# Autodesk Inventor assembly: car
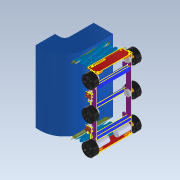
[picture p0: Inventor's stored thumbnail of the model, 180x180]
Saved by Autodesk Inventor 2022 (Build 260153000, 153)
## iProperties
Created: 2023-04-20
Part Number: car
Document SubType Name: Assembly
Designer: Johnny Jou
Author: Johnny Jou
## Documents named in this file (24)
- C:\Users\Johnny Jou\Documents\GitHub\Areo_Rider_Cabin\car\car.iam
- C:\Users\Johnny Jou\Documents\GitHub\Areo_Rider_Cabin\car\chassis_1_1\chassis_1_1-02.ipt
- C:\Users\Johnny Jou\Documents\GitHub\Areo_Rider_Cabin\car\chassis_1_1.ipt
- C:\Users\Johnny Jou\Documents\GitHub\Areo_Rider_Cabin\car\chassis_1_1\chassis_1_1-03.ipt
- C:\Users\Johnny Jou\Documents\GitHub\Areo_Rider_Cabin\car\chassis_1_2.ipt
- C:\Users\Johnny Jou\Documents\GitHub\Areo_Rider_Cabin\Expansion\link_2022.ipt
- C:\Users\Johnny Jou\Documents\GitHub\Areo_Rider_Cabin\Expansion\gasket.ipt
- C:\Users\Johnny Jou\Documents\GitHub\Areo_Rider_Cabin\car\car\機械便覽魔法師\軸承1.iam
- C:\Users\Johnny Jou\Documents\GitHub\Areo_Rider_Cabin\car\wheel_base_cover.ipt
- C:\Users\Johnny Jou\Documents\GitHub\Areo_Rider_Cabin\car\axle 4_20.ipt
- C:\Users\Johnny Jou\Documents\GitHub\Areo_Rider_Cabin\car\Coupling.ipt
- C:\Users\Johnny Jou\Documents\GitHub\Areo_Rider_Cabin\car\wheel.ipt
- C:\Users\Johnny Jou\Documents\GitHub\Areo_Rider_Cabin\car\外抓檔\25GA370.ipt
- C:\Users\Johnny Jou\Documents\GitHub\Areo_Rider_Cabin\Expansion\rod_2.ipt
- C:\Users\Johnny Jou\Documents\GitHub\Areo_Rider_Cabin\car\chassis_1_4.ipt
- C:\Users\Johnny Jou\Documents\GitHub\Areo_Rider_Cabin\car\motorbase_1.ipt
- C:\Users\Johnny Jou\Documents\GitHub\Areo_Rider_Cabin\car\motorbase_2.ipt
- C:\Users\Johnny Jou\Documents\GitHub\Areo_Rider_Cabin\car\motorbase_3.ipt
- C:\Users\Johnny Jou\Documents\GitHub\Areo_Rider_Cabin\car\motorbase_4.ipt
- C:\Users\Johnny Jou\Documents\GitHub\Areo_Rider_Cabin\car\外抓檔\GA12-N20 Motor-Complet.iam
- C:\Users\Johnny Jou\Documents\GitHub\Areo_Rider_Cabin\car\motorbase_5.ipt
- C:\Users\Johnny Jou\Documents\GitHub\Areo_Rider_Cabin\car\chassis_1_2_up.ipt
- C:\Users\Johnny Jou\Documents\GitHub\Areo_Rider_Cabin\car\chassis_1_3.ipt
- C:\Users\Johnny Jou\Documents\GitHub\Areo_Rider_Cabin\Airfoil & Nuzzle\nuzzle\nuzzle_v2_0327.ipt
## Components (76 placed, 22 different names)
1. chassis_1_1-02:1 — 齊平:1, 貼合:4, 貼合:5, 齊平:3, 貼合:6, 貼合:7, 貼合:46, 貼合:47, 貼合:48, 貼合:59, 貼合:60, 貼合:61, 貼合:68, 貼合:69, 貼合:70, 齊平:12, 齊平:21, 貼合:112, 貼合:113, 貼合:114, 貼合:115, 貼合:116, 齊平:32, 貼合:117, 齊平:33, 貼合:118, 貼合:119, 齊平:34, 貼合:120, 貼合:121, 齊平:35, 貼合:122
2. chassis_1_1-03:2 — 貼合:2, 貼合:3, 齊平:2, 貼合:43, 貼合:44, 貼合:45, 貼合:56, 貼合:57, 貼合:58, 貼合:71, 貼合:72, 貼合:73, 齊平:14, 齊平:18, 貼合:83, 貼合:84, 貼合:85, 貼合:86, 貼合:87, 貼合:88, 貼合:89, 貼合:90, 貼合:94, 貼合:96, 貼合:97, 貼合:103, 貼合:104, 貼合:105, 貼合:106, 貼合:107, 貼合:108, 貼合:109
3. chassis_1_2:1 — 齊平:1, 貼合:2, 貼合:3, 齊平:2, 貼合:4, 貼合:5, 插入:16, 貼合:8, 角度:7, 貼合:82, 齊平:11, 齊平:15
4. chassis_1_2:2 — 齊平:3, 貼合:6, 貼合:7, 插入:17, 貼合:9, 齊平:17, 齊平:20
5. link_2022:1 — 插入:1, 插入:3, 角度:1, 插入:17
6. link_2022:2 — 插入:1, 插入:2, 插入:7, 角度:2
7. link_2022:3 — 插入:2, 插入:4, 插入:6, 角度:2
8. link_2022:4 — 插入:3, 插入:4, 角度:1, 貼合:9, 貼合:80, 貼合:81
9. link_2022:5 — 插入:6, 角度:3, 插入:21
10. link_2022:6 — 插入:7, 角度:3, 貼合:110
11. link_2022:7 — 貼合:8, 插入:18
12. link_2022:8
13. link_2022:9
14. link_2022:10 — 插入:15
15. link_2022:11 — 貼合:111
16. link_2022:12 — 插入:22
17. gasket:1 — 插入:15, 插入:16
18. 軸承:2 [sub-assembly]
19. wheel_base_cover:2 — 貼合:43, 貼合:44, 貼合:45
20. axle 4_20:2
21. Coupling:2
22. wheel:2
23. 軸承:3 [sub-assembly]
24. wheel_base_cover:3 — 貼合:46, 貼合:47, 貼合:48
25. axle 4_20:3
26. Coupling:3
27. wheel:3
28. 軸承:4 [sub-assembly]
29. wheel_base_cover:4 — 貼合:59, 貼合:60, 貼合:61
30. axle 4_20:4
31. Coupling:4
32. wheel:4 — 齊平:36
33. Coupling:5 — 貼合:62, 貼合:63
34. wheel:5
35. 軸承:5 [sub-assembly]
36. wheel_base_cover:5 — 貼合:56, 貼合:57, 貼合:58
37. axle 4_20:5
38. Coupling:6
39. wheel:6
40. 25GA370:1 — 貼合:62, 貼合:63, 貼合:71, 貼合:72, 貼合:73
41. Coupling:7
42. wheel:7
43. 25GA370:2 — 貼合:68, 貼合:69, 貼合:70
44. rod_2:1 — 貼合:75, 貼合:76, 貼合:78, 貼合:79, 角度:7, 貼合:80, 貼合:81
45. 軸承:6 [sub-assembly] — 貼合:76
46. axle 4_20:8 — 貼合:75
47. 軸承:7 [sub-assembly] — 貼合:79
48. axle 4_20:9 — 貼合:78
49. gasket:2 — 插入:18
50. chassis_1_4:1 — 貼合:82, 齊平:11, 齊平:12, 齊平:13, 齊平:16, 齊平:19
51. chassis_1_4:2 — 齊平:19, 齊平:20, 齊平:21
52. chassis_1_4:3 — 齊平:16, 齊平:17, 齊平:18
53. chassis_1_4:4 — 齊平:13, 齊平:14, 齊平:15
54. motorbase_1:1 — 貼合:88, 貼合:89, 貼合:90, 齊平:25
55. motorbase_2:1 — 貼合:83, 貼合:84, 貼合:85, 齊平:22, 貼合:93, 貼合:95
56. motorbase_3:1 — 齊平:25, 貼合:96, 貼合:97
57. motorbase_4:1 — 插入:19, 齊平:23, 齊平:24
58. GA12-N20 Motor-Complet:1 [sub-assembly] — 貼合:91, 貼合:92, 齊平:24, 貼合:93, 貼合:94, 貼合:95
59. motorbase_2:2 — 貼合:86, 貼合:87, 齊平:22
60. motorbase_5:1 — 插入:19, 齊平:23, 貼合:91, 貼合:92
61. motorbase_1:2 — 齊平:31, 貼合:106, 貼合:107
62. motorbase_2:3 — 齊平:30, 齊平:31, 貼合:105
63. motorbase_3:2 — 貼合:108, 貼合:109
64. motorbase_4:2
65. GA12-N20 Motor-Complet:2 [sub-assembly] — 貼合:102
66. motorbase_2:4 — 齊平:30, 貼合:102, 貼合:103, 貼合:104
67. motorbase_5:2
68. chassis_1_2_up:1 — 插入:21, 貼合:110, 貼合:123
69. chassis_1_2_up:2 — 插入:23, 貼合:111, 齊平:37
70. gasket:3 — 插入:22, 插入:23
71. chassis_1_3:1 — 貼合:115, 貼合:116, 齊平:32
72. chassis_1_3:2 — 貼合:112, 貼合:113, 貼合:114
73. chassis_1_3:3 — 貼合:117, 齊平:33, 貼合:118
74. chassis_1_3:4 — 貼合:119, 齊平:34, 貼合:120
75. chassis_1_3:5 — 貼合:121, 齊平:35, 貼合:122
76. nuzzle_v2_0327:1 — 貼合:123, 齊平:36, 齊平:37
## Relationships (178: Mate 112, Flush 36, Insert 23, Angle 7)
- 齊平:1 [Flush]: chassis_1_1-02:1 ↔ chassis_1_2:1
- 貼合:2 [Mate]: chassis_1_1-03:2 ↔ chassis_1_2:1
- 貼合:3 [Mate]: chassis_1_1-03:2 ↔ chassis_1_2:1
- 齊平:2 [Flush]: chassis_1_1-03:2 ↔ chassis_1_2:1
- 貼合:4 [Mate]: chassis_1_1-02:1 ↔ chassis_1_2:1
- 貼合:5 [Mate]: chassis_1_1-02:1 ↔ chassis_1_2:1
- 齊平:3 [Flush]: chassis_1_1-02:1 ↔ chassis_1_2:2
- 貼合:6 [Mate]: chassis_1_1-02:1 ↔ chassis_1_2:2
- 貼合:7 [Mate]: chassis_1_1-02:1 ↔ chassis_1_2:2
- 插入:1 [Insert]: link_2022:1 ↔ link_2022:2
- 插入:2 [Insert]: link_2022:2 ↔ link_2022:3
- 插入:3 [Insert]: link_2022:1 ↔ link_2022:4
- 插入:4 [Insert]: link_2022:3 ↔ link_2022:4
- [Insert]: link_2022:5 ↔ link_2022:6
- 插入:6 [Insert]: link_2022:3 ↔ link_2022:5
- 插入:7 [Insert]: link_2022:2 ↔ link_2022:6
- 角度:1 [Angle] (20 deg): link_2022:1 ↔ link_2022:4
- 角度:2 [Angle] (20 deg): link_2022:2 ↔ link_2022:3
- 角度:3 [Angle] (20 deg): link_2022:5 ↔ link_2022:6
- [Insert]: link_2022:7 ↔ link_2022:8
- [Insert]: link_2022:8 ↔ link_2022:9
- [Insert]: link_2022:7 ↔ link_2022:10
- [Insert]: link_2022:9 ↔ link_2022:10
- [Insert]: link_2022:11 ↔ link_2022:12
- [Insert]: link_2022:9 ↔ link_2022:11
- [Insert]: link_2022:8 ↔ link_2022:12
- [Angle] (20 deg): link_2022:7 ↔ link_2022:10
- [Angle] (20 deg): link_2022:8 ↔ link_2022:9
- [Angle] (20 deg): link_2022:11 ↔ link_2022:12
- 插入:15 [Insert]: link_2022:10 ↔ gasket:1
- 插入:16 [Insert]: chassis_1_2:1 ↔ gasket:1
- 貼合:8 [Mate]: chassis_1_2:1 ↔ link_2022:7
- 插入:17 [Insert]: chassis_1_2:2 ↔ link_2022:1
- 貼合:9 [Mate]: chassis_1_2:2 ↔ link_2022:4
- [Mate]: 軸承:2 ↔ wheel_base_cover:2
- [Mate]: 軸承:2 ↔ wheel_base_cover:2
- [Mate]: 軸承:2 ↔ axle 4_20:2
- [Flush]: 軸承:2 ↔ axle 4_20:2
- [Mate]: axle 4_20:2 ↔ Coupling:2
- [Mate] (5 mm): wheel_base_cover:2 ↔ Coupling:2
- [Mate]: Coupling:2 ↔ wheel:2
- [Mate]: Coupling:2 ↔ wheel:2
- [Mate]: 軸承:3 ↔ wheel_base_cover:3
- [Mate]: 軸承:3 ↔ wheel_base_cover:3
- [Mate]: 軸承:3 ↔ axle 4_20:3
- [Flush]: 軸承:3 ↔ axle 4_20:3
- [Mate]: axle 4_20:3 ↔ Coupling:3
- [Mate] (5 mm): wheel_base_cover:3 ↔ Coupling:3
- [Mate]: Coupling:3 ↔ wheel:3
- [Mate]: Coupling:3 ↔ wheel:3
- [Mate]: 軸承:4 ↔ wheel_base_cover:4
- [Mate]: 軸承:4 ↔ wheel_base_cover:4
- [Mate]: 軸承:4 ↔ axle 4_20:4
- [Flush]: 軸承:4 ↔ axle 4_20:4
- [Mate]: axle 4_20:4 ↔ Coupling:4
- [Mate] (5 mm): wheel_base_cover:4 ↔ Coupling:4
- [Mate]: Coupling:4 ↔ wheel:4
- [Mate]: Coupling:4 ↔ wheel:4
- [Mate]: Coupling:5 ↔ wheel:5
- [Mate]: Coupling:5 ↔ wheel:5
- 貼合:43 [Mate]: chassis_1_1-03:2 ↔ wheel_base_cover:2
- 貼合:44 [Mate]: chassis_1_1-03:2 ↔ wheel_base_cover:2
- 貼合:45 [Mate]: chassis_1_1-03:2 ↔ wheel_base_cover:2
- 貼合:46 [Mate]: chassis_1_1-02:1 ↔ wheel_base_cover:3
- 貼合:47 [Mate]: chassis_1_1-02:1 ↔ wheel_base_cover:3
- 貼合:48 [Mate]: chassis_1_1-02:1 ↔ wheel_base_cover:3
- [Mate]: 軸承:5 ↔ wheel_base_cover:5
- [Mate]: 軸承:5 ↔ wheel_base_cover:5
- [Mate]: 軸承:5 ↔ axle 4_20:5
- [Flush]: 軸承:5 ↔ axle 4_20:5
- [Mate]: axle 4_20:5 ↔ Coupling:6
- [Mate] (5 mm): wheel_base_cover:5 ↔ Coupling:6
- [Mate]: Coupling:6 ↔ wheel:6
- [Mate]: Coupling:6 ↔ wheel:6
- 貼合:56 [Mate]: chassis_1_1-03:2 ↔ wheel_base_cover:5
- 貼合:57 [Mate]: chassis_1_1-03:2 ↔ wheel_base_cover:5
- 貼合:58 [Mate]: chassis_1_1-03:2 ↔ wheel_base_cover:5
- 貼合:59 [Mate]: chassis_1_1-02:1 ↔ wheel_base_cover:4
- 貼合:60 [Mate]: chassis_1_1-02:1 ↔ wheel_base_cover:4
- 貼合:61 [Mate]: chassis_1_1-02:1 ↔ wheel_base_cover:4
- 貼合:62 [Mate]: Coupling:5 ↔ 25GA370:1
- 貼合:63 [Mate] (5 mm): Coupling:5 ↔ 25GA370:1
- [Mate]: Coupling:7 ↔ wheel:7
- [Mate]: Coupling:7 ↔ wheel:7
- [Mate]: Coupling:7 ↔ 25GA370:2
- [Mate] (5 mm): Coupling:7 ↔ 25GA370:2
- 貼合:68 [Mate]: chassis_1_1-02:1 ↔ 25GA370:2
- 貼合:69 [Mate]: chassis_1_1-02:1 ↔ 25GA370:2
- 貼合:70 [Mate]: chassis_1_1-02:1 ↔ 25GA370:2
- 貼合:71 [Mate]: chassis_1_1-03:2 ↔ 25GA370:1
- 貼合:72 [Mate]: chassis_1_1-03:2 ↔ 25GA370:1
- 貼合:73 [Mate]: chassis_1_1-03:2 ↔ 25GA370:1
- [Mate]: 軸承:6 ↔ axle 4_20:8
- [Flush]: 軸承:6 ↔ axle 4_20:8
- 貼合:75 [Mate]: rod_2:1 ↔ axle 4_20:8
- 貼合:76 [Mate]: rod_2:1 ↔ 軸承:6
- [Mate]: 軸承:7 ↔ axle 4_20:9
- [Flush]: 軸承:7 ↔ axle 4_20:9
- 貼合:78 [Mate]: rod_2:1 ↔ axle 4_20:9
- 貼合:79 [Mate]: rod_2:1 ↔ 軸承:7
- 角度:7 [Angle] (0 deg): chassis_1_2:1 ↔ rod_2:1
- 貼合:80 [Mate]: link_2022:4 ↔ rod_2:1
- 貼合:81 [Mate]: link_2022:4 ↔ rod_2:1
- 插入:18 [Insert]: link_2022:7 ↔ gasket:2
- 貼合:82 [Mate]: chassis_1_2:1 ↔ chassis_1_4:1
- 齊平:11 [Flush]: chassis_1_2:1 ↔ chassis_1_4:1
- 齊平:12 [Flush]: chassis_1_1-02:1 ↔ chassis_1_4:1
- 齊平:13 [Flush]: chassis_1_4:1 ↔ chassis_1_4:4
- 齊平:14 [Flush]: chassis_1_1-03:2 ↔ chassis_1_4:4
- 齊平:15 [Flush]: chassis_1_2:1 ↔ chassis_1_4:4
- 齊平:16 [Flush]: chassis_1_4:1 ↔ chassis_1_4:3
- 齊平:17 [Flush]: chassis_1_2:2 ↔ chassis_1_4:3
- 齊平:18 [Flush]: chassis_1_1-03:2 ↔ chassis_1_4:3
- 齊平:19 [Flush]: chassis_1_4:1 ↔ chassis_1_4:2
- 齊平:20 [Flush]: chassis_1_2:2 ↔ chassis_1_4:2
- 齊平:21 [Flush]: chassis_1_1-02:1 ↔ chassis_1_4:2
- 貼合:83 [Mate]: chassis_1_1-03:2 ↔ motorbase_2:1
- 貼合:84 [Mate]: chassis_1_1-03:2 ↔ motorbase_2:1
- 貼合:85 [Mate]: chassis_1_1-03:2 ↔ motorbase_2:1
- 貼合:86 [Mate]: chassis_1_1-03:2 ↔ motorbase_2:2
- 貼合:87 [Mate]: chassis_1_1-03:2 ↔ motorbase_2:2
- 齊平:22 [Flush]: motorbase_2:1 ↔ motorbase_2:2
- 貼合:88 [Mate]: chassis_1_1-03:2 ↔ motorbase_1:1
- 貼合:89 [Mate]: chassis_1_1-03:2 ↔ motorbase_1:1
- 貼合:90 [Mate]: chassis_1_1-03:2 ↔ motorbase_1:1
- 插入:19 [Insert]: motorbase_4:1 ↔ motorbase_5:1
- 齊平:23 [Flush]: motorbase_4:1 ↔ motorbase_5:1
- 貼合:91 [Mate]: GA12-N20 Motor-Complet:1 ↔ motorbase_5:1
- 貼合:92 [Mate]: GA12-N20 Motor-Complet:1 ↔ motorbase_5:1
- 齊平:24 [Flush]: motorbase_4:1 ↔ GA12-N20 Motor-Complet:1
- 貼合:93 [Mate]: motorbase_2:1 ↔ GA12-N20 Motor-Complet:1
- 貼合:94 [Mate]: chassis_1_1-03:2 ↔ GA12-N20 Motor-Complet:1
- 貼合:95 [Mate]: motorbase_2:1 ↔ GA12-N20 Motor-Complet:1
- 齊平:25 [Flush]: motorbase_1:1 ↔ motorbase_3:1
- 貼合:96 [Mate]: chassis_1_1-03:2 ↔ motorbase_3:1
- 貼合:97 [Mate]: chassis_1_1-03:2 ↔ motorbase_3:1
- [Flush]: motorbase_2:3 ↔ motorbase_2:4
- [Insert]: motorbase_4:2 ↔ motorbase_5:2
- [Flush]: motorbase_4:2 ↔ motorbase_5:2
- [Mate]: GA12-N20 Motor-Complet:2 ↔ motorbase_5:2
- [Mate]: GA12-N20 Motor-Complet:2 ↔ motorbase_5:2
- [Flush]: motorbase_4:2 ↔ GA12-N20 Motor-Complet:2
- [Mate]: motorbase_2:3 ↔ GA12-N20 Motor-Complet:2
- [Mate]: motorbase_2:3 ↔ GA12-N20 Motor-Complet:2
- [Flush]: motorbase_1:2 ↔ motorbase_3:2
- 齊平:30 [Flush]: motorbase_2:3 ↔ motorbase_2:4
- 貼合:102 [Mate]: GA12-N20 Motor-Complet:2 ↔ motorbase_2:4
- 齊平:31 [Flush]: motorbase_1:2 ↔ motorbase_2:3
- 貼合:103 [Mate]: chassis_1_1-03:2 ↔ motorbase_2:4
- 貼合:104 [Mate]: chassis_1_1-03:2 ↔ motorbase_2:4
- 貼合:105 [Mate]: chassis_1_1-03:2 ↔ motorbase_2:3
- 貼合:106 [Mate]: chassis_1_1-03:2 ↔ motorbase_1:2
- 貼合:107 [Mate]: chassis_1_1-03:2 ↔ motorbase_1:2
- 貼合:108 [Mate]: chassis_1_1-03:2 ↔ motorbase_3:2
- 貼合:109 [Mate]: chassis_1_1-03:2 ↔ motorbase_3:2
- 插入:21 [Insert]: link_2022:5 ↔ chassis_1_2_up:1
- 貼合:110 [Mate]: link_2022:6 ↔ chassis_1_2_up:1
- 插入:22 [Insert]: link_2022:12 ↔ gasket:3
- 插入:23 [Insert]: chassis_1_2_up:2 ↔ gasket:3
- 貼合:111 [Mate]: link_2022:11 ↔ chassis_1_2_up:2
- 貼合:112 [Mate]: chassis_1_1-02:1 ↔ chassis_1_3:2
- 貼合:113 [Mate]: chassis_1_1-02:1 ↔ chassis_1_3:2
- 貼合:114 [Mate]: chassis_1_1-02:1 ↔ chassis_1_3:2
- 貼合:115 [Mate]: chassis_1_1-02:1 ↔ chassis_1_3:1
- 貼合:116 [Mate]: chassis_1_1-02:1 ↔ chassis_1_3:1
- 齊平:32 [Flush]: chassis_1_1-02:1 ↔ chassis_1_3:1
- 貼合:117 [Mate]: chassis_1_1-02:1 ↔ chassis_1_3:3
- 齊平:33 [Flush]: chassis_1_1-02:1 ↔ chassis_1_3:3
- 貼合:118 [Mate]: chassis_1_1-02:1 ↔ chassis_1_3:3
- 貼合:119 [Mate]: chassis_1_1-02:1 ↔ chassis_1_3:4
- 齊平:34 [Flush]: chassis_1_1-02:1 ↔ chassis_1_3:4
- 貼合:120 [Mate]: chassis_1_1-02:1 ↔ chassis_1_3:4
- 貼合:121 [Mate]: chassis_1_1-02:1 ↔ chassis_1_3:5
- 齊平:35 [Flush]: chassis_1_1-02:1 ↔ chassis_1_3:5
- 貼合:122 [Mate]: chassis_1_1-02:1 ↔ chassis_1_3:5
- 貼合:123 [Mate]: chassis_1_2_up:1 ↔ nuzzle_v2_0327:1
- 齊平:36 [Flush]: wheel:4 ↔ nuzzle_v2_0327:1
- 齊平:37 [Flush] (-12 mm): chassis_1_2_up:2 ↔ nuzzle_v2_0327:1
## Named parameters: d14_d11 = 0 mm, d20_d10 = 0 mm, d21_d11 = 0 mm, d22_d12 = 0 mm, d23_d13 = 0 mm, d24_d14_d11 = 0 mm, d25_d15 = 0 mm, d26_d16 = 0 mm, d27_d17 = 20 deg, d28_d18 = 20 deg, d29_d19 = 20 deg, d49_d41 = 0 mm, d50_d42 = 0 mm, d51_d43 = 0 mm, d52_d44 = 0 mm, d53_d45 = 0 mm, d54_d46 = 5 mm, d55_d47 = 0 mm, d56_d48 = 0 mm, d57_d41 = 0 mm, d58_d42 = 0 mm, d59_d43 = 0 mm, d60_d44 = 0 mm, d61_d45 = 0 mm, d62_d46 = 5 mm, d63_d47 = 0 mm, d64_d48 = 0 mm, d65_d41 = 0 mm, d66_d42 = 0 mm, d67_d43 = 0 mm, d68_d44 = 0 mm, d69_d45 = 0 mm, d70_d46 = 5 mm, d71_d47 = 0 mm, d72_d48 = 0 mm, d73_d55_d47 = 0 mm, d74_d56_d48 = 0 mm, d84_d65_d41 = 0 mm, d85_d66_d42 = 0 mm, d86_d67_d43 = 0 mm, d87_d68_d44 = 0 mm, d88_d69_d45 = 0 mm, d89_d70_d46 = 5 mm, d90_d71_d47 = 0 mm, d91_d72_d48 = 0 mm, d100_d98 = 0 mm, d101_d99 = 5 mm, d102_d73_d55_d47 = 0 mm, d103_d74_d56_d48 = 0 mm, d110_d59_d43 = 0 mm, d111_d60_d44 = 0 mm, d114_d110_d59_d43 = 0 mm, d115_d111_d60_d44 = 0 mm, d156_d145 = 0 mm, d157_d146 = 0 mm, d158_d147 = 0 mm, d159_d148 = 0 mm, d160_d149 = 0 mm, d161_d150 = 0 mm, d162_d152 = 0 mm, d163_d153 = 0 mm, d164_d140 = 0 mm
